# Autodesk Inventor assembly: Default Motor Testbench Mk4
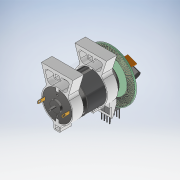
[picture p0: Inventor's stored thumbnail of the model, 180x180]
Saved by Autodesk Inventor 2018.2 (Build 222227000, 227)
## iProperties
Created: 2018-01-25
Part Number: Default Motor Testbench Mk4
Document SubType Name: Assembly
Designer: Moochster
Author: Moochster
## Documents named in this file (10)
- C:\Users\Moochster\OneDrive\Documents\2018 UBC\ELEC 391\Controller\CAD\Default Motor Testbench Mk4.iam
- C:\Users\Moochster\OneDrive\Documents\2018 UBC\ELEC 391\Controller\CAD\JD5B-2655W-R.ipt
- C:\Users\Moochster\OneDrive\Documents\2018 UBC\ELEC 391\Controller\CAD\Encoder Wheel (G16).ipt
- C:\Users\Moochster\OneDrive\Documents\2018 UBC\ELEC 391\Controller\CAD\Laser Mount.ipt
- C:\Users\Moochster\OneDrive\Documents\2018 UBC\ELEC 391\Controller\CAD\Motor Reversed Mount.ipt
- C:\Users\Moochster\OneDrive\Documents\2018 UBC\ELEC 391\Controller\CAD\Motor Reversed Mount Midsection.ipt
- C:\Users\Moochster\OneDrive\Documents\2018 UBC\ELEC 391\Controller\CAD\Motor Mount Slot Lock.ipt
- C:\Users\Moochster\OneDrive\Documents\2018 UBC\ELEC 391\Controller\CAD\GP1A52HRJ00F (Large slot detector).ipt
- C:\Users\Moochster\OneDrive\Documents\2018 UBC\ELEC 391\Controller\CAD\VLM-650-03-LPT.ipt
- C:\Users\Moochster\OneDrive\Documents\2018 UBC\ELEC 391\Controller\CAD\Encoder Mount.ipt
## Components (11 placed, 9 different names)
1. JD5B-2655W-R:1 — Mate:1, Mate:2, Mate:3, Mate:5, Flush:2, Mate:6, Mate:13
2. Encoder Wheel (G16):1 — Mate:1, Mate:12, Mate:13, Angle:3, Mate:17
3. Laser Mount:1 — Mate:2, Angle:3, Mate:17, Mate:18, Flush:6
4. Motor Reversed Mount:1 — Mate:5, Angle:1, Flush:2, Flush:3, Mate:7, Mate:8, Mate:9, Mate:10
5. Motor Reversed Mount Midsection:1 — Mate:6, Flush:3
6. Motor Mount Slot Lock:1 — Mate:7, Mate:8
7. Motor Mount Slot Lock:2 — Mate:9, Mate:10
8. GP1A52HRJ00F (Large slot detector):1 — Mate:11, Flush:4, Flush:5, Angle:2, Mate:16, Mate:20, Flush:7
9. GP1A52HRJ00F (Large slot detector):2 — Mate:11, Flush:4, Flush:5, Mate:12, Mate:19
10. VLM-650-03-LPT:1 — Mate:18, Flush:6
11. Encoder Mount:1 — Mate:19, Mate:20, Flush:7
## Relationships (26: Mate 17, Flush 6, Angle 3)
- Mate:1: JD5B-2655W-R:1 ↔ Encoder Wheel (G16):1
- Mate:2: JD5B-2655W-R:1 ↔ Laser Mount:1
- Mate:3: JD5B-2655W-R:1
- Mate:5: JD5B-2655W-R:1 ↔ Motor Reversed Mount:1
- Angle:1 (0 deg): Motor Reversed Mount:1
- Flush:2: JD5B-2655W-R:1 ↔ Motor Reversed Mount:1
- Mate:6: JD5B-2655W-R:1 ↔ Motor Reversed Mount Midsection:1
- Flush:3: Motor Reversed Mount:1 ↔ Motor Reversed Mount Midsection:1
- Mate:7 (0.15 mm): Motor Reversed Mount:1 ↔ Motor Mount Slot Lock:1
- Mate:8 (0.15 mm): Motor Reversed Mount:1 ↔ Motor Mount Slot Lock:1
- Mate:9 (0.15 mm): Motor Reversed Mount:1 ↔ Motor Mount Slot Lock:2
- Mate:10 (0.15 mm): Motor Reversed Mount:1 ↔ Motor Mount Slot Lock:2
- Mate:11 (0.1 mm): GP1A52HRJ00F (Large slot detector):1 ↔ GP1A52HRJ00F (Large slot detector):2
- Flush:4: GP1A52HRJ00F (Large slot detector):1 ↔ GP1A52HRJ00F (Large slot detector):2
- Flush:5: GP1A52HRJ00F (Large slot detector):1 ↔ GP1A52HRJ00F (Large slot detector):2
- Mate:12 (0.75 mm): Encoder Wheel (G16):1 ↔ GP1A52HRJ00F (Large slot detector):2
- Angle:2 (0 deg): GP1A52HRJ00F (Large slot detector):1
- Mate:13 (1 mm): JD5B-2655W-R:1 ↔ Encoder Wheel (G16):1
- Angle:3 (0 deg): Encoder Wheel (G16):1 ↔ Laser Mount:1
- Mate:16: GP1A52HRJ00F (Large slot detector):1
- Mate:17 (1 mm): Encoder Wheel (G16):1 ↔ Laser Mount:1
- Mate:18: Laser Mount:1 ↔ VLM-650-03-LPT:1
- Flush:6 (-6 mm): Laser Mount:1 ↔ VLM-650-03-LPT:1
- Mate:19 (0.15 mm): GP1A52HRJ00F (Large slot detector):2 ↔ Encoder Mount:1
- Mate:20 (0.2 mm): GP1A52HRJ00F (Large slot detector):1 ↔ Encoder Mount:1
- Flush:7: GP1A52HRJ00F (Large slot detector):1 ↔ Encoder Mount:1
